# Autodesk Inventor assembly: V2 modular session micro cam adj mount 45 deg
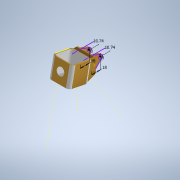
[picture p0: Inventor's stored thumbnail of the model, 180x180]
Saved by Autodesk Inventor 2020 (Build 240168000, 168)
## iProperties
Created: 2022-08-01
Part Number: V2 modular session micro cam adj mount 45 deg
Document SubType Name: Assembly
Designer: Steven
Author: Steven
## Documents named in this file (3)
- Y:\FPV drone stuff\0 Street League\Frames\PB-Kauri-X\3D prints\35 mm canopy\work in progress prints\session mounts\V2 modular session micro cam adj mount 45 deg.iam
- Y:\FPV drone stuff\0 Street League\Frames\PB-Kauri-X\3D prints\35 mm canopy\work in progress prints\session mounts\V2 session mount 45deg block.ipt
- Y:\FPV drone stuff\0 Street League\Frames\PB-Kauri-X\3D prints\35 mm canopy\work in progress prints\Camera mounts\Kauri modular camera mount HDzero micro v1.ipt
## Components (3 placed, 2 different names)
1. V2 session mount 45deg block:1 — Flush:1, Flush:2, Flush:3, Mate:1, Flush:4, Flush:5, Flush:6, Mate:2, Mate:3, Mate:4, Flush:7
2. Kauri modular camera mount HDzero micro v1:1 — Mate:3, Mate:4, Mate:5
3. Kauri modular camera mount HDzero micro v1:2 — Mate:1, Mate:2, Mate:5, Flush:7
## Relationships (12: Flush 7, Mate 5)
- Flush:1: V2 session mount 45deg block:1
- Flush:2: V2 session mount 45deg block:1
- Flush:3: V2 session mount 45deg block:1
- Mate:1: V2 session mount 45deg block:1 ↔ Kauri modular camera mount HDzero micro v1:2
- Flush:4: V2 session mount 45deg block:1
- Flush:5: V2 session mount 45deg block:1
- Flush:6: V2 session mount 45deg block:1
- Mate:2: V2 session mount 45deg block:1 ↔ Kauri modular camera mount HDzero micro v1:2
- Mate:3: V2 session mount 45deg block:1 ↔ Kauri modular camera mount HDzero micro v1:1
- Mate:4: V2 session mount 45deg block:1 ↔ Kauri modular camera mount HDzero micro v1:1
- Mate:5 (19.1 mm): Kauri modular camera mount HDzero micro v1:1 ↔ Kauri modular camera mount HDzero micro v1:2
- Flush:7 (3.95 mm): V2 session mount 45deg block:1 ↔ Kauri modular camera mount HDzero micro v1:2
